# Autodesk Inventor assembly: Rail_AssemblyV2_0
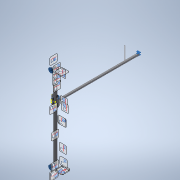
[picture p0: Inventor's stored thumbnail of the model, 180x180]
Saved by Autodesk Inventor 2021 (Build 250183000, 183)
## iProperties
Created: 2021-01-25
Part Number: Rail_AssemblyV2_0
Document SubType Name: Assembly
Designer: Jorian Brusind
Mass: 3786.54 g
Surface Area: 19508.5 cm^2
Volume: 2323.9 cm^3
Density: 1.62939 g/cm^3
Author: Jorian Brusind
## Documents named in this file (33)
- C:\Users\Jorian Brusind\Documents\GitHub\PersonalProjects\HyperRail\Inventor Files\Rail_AssemblyV2_0.iam
- C:\Users\Jorian Brusind\Documents\GitHub\PersonalProjects\Inventor Projects\Useful models\NEMA_Steppers\NEMA23\23HS8430B.ipt
- C:\Users\Jorian Brusind\Documents\GitHub\PersonalProjects\HyperRail\Inventor Files\NEMA23_StepperonlineMount.ipt
- C:\Users\Jorian Brusind\Documents\GitHub\PersonalProjects\Inventor Projects\Useful models\8020_Sets\IPT_20_Series\IPT_20_Series\20-2040_200mm.ipt
- C:\Users\Jorian Brusind\Documents\GitHub\PersonalProjects\HyperRail\Inventor Files\2804S_NEMA2115_1Gearbox.ipt
- C:\Users\Jorian Brusind\Documents\GitHub\PersonalProjects\HyperRail\PCB Files\Integrated Stepper Motor Driver\ExportSTEP\Main.iam
- C:\Users\Jorian Brusind\Documents\GitHub\PersonalProjects\HyperRail\Inventor Files\NEMA23_Shroud.ipt
- C:\Users\Jorian Brusind\Documents\GitHub\PersonalProjects\Inventor Projects\Useful models\8020_Sets\IPT_20_Series\IPT_20_Series\20-4040_2m.ipt
- C:\Users\Jorian Brusind\Documents\GitHub\PersonalProjects\HyperRail\Inventor Files\98952A059_ALUM MALE-FEM THRDED HEX STANDOFF.ipt
- C:\Users\Jorian Brusind\Documents\GitHub\PersonalProjects\HyperRail\Inventor Files\95783A039_NYLON 6-6 MALE-FEM THRDED HEX STANDOFF.ipt
- C:\Users\Jorian Brusind\Documents\GitHub\PersonalProjects\HyperRail\Inventor Files\Integrated_Stepper_NEMA23_Mount.ipt
- C:\Users\Jorian Brusind\Documents\GitHub\PersonalProjects\HyperRail\Inventor Files\Foot_Spacer.ipt
- C:\Users\Jorian Brusind\Documents\GitHub\PersonalProjects\Inventor Projects\Useful models\Metric bolt\Bolt M5 50mm.ipt
- C:\Users\Jorian Brusind\Documents\GitHub\PersonalProjects\Inventor Projects\Useful models\Metric nuts\Nut M5.ipt
- C:\Users\Jorian Brusind\Documents\GitHub\PersonalProjects\HyperRail\Inventor Files\Bottom_Foot.ipt
- C:\Users\Jorian Brusind\Documents\GitHub\PersonalProjects\HyperRail\Inventor Files\90deg_4040Bracket.ipt
- C:\Users\Jorian Brusind\Documents\GitHub\PersonalProjects\HyperRail\Inventor Files\X_Carriage_V2_0.iam
- C:\Users\Jorian Brusind\Documents\GitHub\PersonalProjects\Inventor Projects\Useful models\8020_Sets\IPT_40_Series\Extra_40_Series\HFS5-4060-4000\HFS5-4060-2125.ipt
- C:\Users\Jorian Brusind\Documents\GitHub\PersonalProjects\Inventor Projects\Useful models\8020_Sets\IPT_20_Series\IPT_20_Series\20-2040_150mm.ipt
- C:\Users\Jorian Brusind\Documents\GitHub\PersonalProjects\HyperRail\Inventor Files\RightAngle_Bracket_60mm.ipt
- C:\Users\Jorian Brusind\Documents\GitHub\PersonalProjects\Inventor Projects\Useful models\e2-micro-e-chains-small-and-lightweight-e-chains\03_07_012_0_160_5.iam
- C:\Users\Jorian Brusind\Documents\GitHub\PersonalProjects\HyperRail\Inventor Files\Cable_Guide_End.ipt
- C:\Users\Jorian Brusind\Documents\GitHub\PersonalProjects\Inventor Projects\Useful models\8020_Sets\AIS2018\20-2568_d.iam
- C:\Users\Jorian Brusind\Documents\GitHub\PersonalProjects\HyperRail\Inventor Files\5mm_bore_10mm_width_idlepulley.ipt
- C:\Users\Jorian Brusind\Documents\GitHub\PersonalProjects\HyperRail\Inventor Files\Idler_Spacer.ipt
- C:\Users\Jorian Brusind\Documents\GitHub\PersonalProjects\HyperRail\Inventor Files\Tape_Belt_Layer.ipt
- C:\Users\Jorian Brusind\Documents\GitHub\PersonalProjects\HyperRail\Inventor Files\SDP_sdpsi_a_6a55m028df0912\SDP_sdpsi_a_6a55m028df0912.ipt
- C:\Users\Jorian Brusind\Documents\GitHub\PersonalProjects\HyperRail\Inventor Files\X_CarriageR_V2_0.iam
- C:\Users\Jorian Brusind\Documents\GitHub\PersonalProjects\HyperRail\Inventor Files\X_CarriageL_V2_0_Short.iam
- C:\Users\Jorian Brusind\Documents\GitHub\PersonalProjects\HyperRail\Inventor Files\X_CarriageR_V2_0_Short.iam
- C:\Users\Jorian Brusind\Documents\GitHub\PersonalProjects\HyperRail\Inventor Files\SDP_sdpsi_a_6r25mc250\SDP_sdpsi_a_6r25mc1000.ipt
- C:\Users\Jorian Brusind\Documents\GitHub\PersonalProjects\Inventor Projects\Useful models\8020_Sets\IPT_20_Series\Extra_20_Series\8020_14056m\14056_m.ipt
- C:\Users\Jorian Brusind\Documents\GitHub\PersonalProjects\HyperRail\Inventor Files\Cable_Guide_Holder.ipt
## Components (51 placed, 32 different names)
1. 23HS8430B:1 — Mate:127, Angle:3, Mate:158, Mate:177, Mate:179, Mate:180, Mate:181, Mate:182, Mate:183, Mate:184, Mate:185, Mate:264, Mate:265, Mate:295
2. NEMA23_StepperonlineMount:1 — Angle:2, Mate:98, Mate:128, Mate:289, Flush:99, Mate:303, Mate:304, Flush:107, Flush:108
3. 20-2040_200mm:1 — Flush:88, Mate:284, Mate:301, Mate:302, Flush:111, Mate:334, Flush:125, Mate:335, Mate:337, Flush:127, Mate:338
4. 2804S_NEMA2115_1Gearbox:1 — Angle:2, Mate:98, Mate:127, Mate:128, Angle:3, Mate:158, Flush:86, Mate:336, Flush:126
5. Main:1 [sub-assembly] — Mate:291, Mate:292, Mate:293
6. 20-4040_2m:2 — Mate:232, Flush:73, Mate:233, Mate:234, Flush:74, Mate:288, Flush:98, Flush:123, Mate:322, Mate:323, Mate:326, Mate:327, Mate:330, Mate:331, Flush:124, Mate:345, Mate:346
7. NEMA23_Shroud:1 — Mate:264, Mate:265, Flush:86, Mate:294
8. 98952A059_ALUM MALE-FEM THRDED HEX STANDOFF:1 — Mate:180, Mate:181, Mate:186, Mate:191
9. 98952A059_ALUM MALE-FEM THRDED HEX STANDOFF:2 — Mate:184, Mate:185, Mate:189, Mate:192
10. 98952A059_ALUM MALE-FEM THRDED HEX STANDOFF:3 — Mate:177, Mate:179, Mate:187, Mate:190
11. 98952A059_ALUM MALE-FEM THRDED HEX STANDOFF:4 — Mate:182, Mate:183, Mate:188, Mate:193
12. 95783A039_NYLON 6-6 MALE-FEM THRDED HEX STANDOFF:1 — Mate:188, Mate:193
13. 95783A039_NYLON 6-6 MALE-FEM THRDED HEX STANDOFF:2 — Mate:186, Mate:191
14. 95783A039_NYLON 6-6 MALE-FEM THRDED HEX STANDOFF:3 — Mate:187, Mate:190
15. 95783A039_NYLON 6-6 MALE-FEM THRDED HEX STANDOFF:4 — Mate:189, Mate:192
16. Bolt M5 50mm:1 — Mate:224, Mate:245, Mate:246, Mate:247, Mate:269
17. Nut M5:1 — Mate:226, Mate:247
18. Nut M5:2 — Mate:244, Flush:78, Mate:246
19. Bottom_Foot:1 — Mate:224, Mate:226, Mate:245, Flush:81, Flush:93
20. 90deg_4040Bracket:1 — Mate:232, Flush:73, Mate:233, Flush:75
21. 90deg_4040Bracket:2 — Mate:234, Flush:74, Flush:75
22. Foot_Spacer:1 — Mate:244, Flush:78, Mate:269, Mate:283, Flush:94
23. Foot_Spacer:2 — Mate:250, Mate:281, Flush:91, Flush:92, Mate:282
24. Bottom_Foot:2 — Mate:249, Mate:251, Flush:81, Flush:93
25. Bolt M5 50mm:2 — Mate:249, Mate:250, Mate:251, Mate:282
26. 20-2040_200mm:2 — Flush:88, Mate:286, Flush:96, Flush:111, Flush:114, Flush:116, Mate:316, Flush:117, Flush:124, Mate:339, Flush:128, Mate:340, Mate:341, Flush:129, Mate:342
27. HFS5-4060-2125:1 — Mate:277, Mate:278, Mate:279, Mate:280, Mate:281, Flush:91, Flush:92, Mate:283, Flush:94, Mate:284, Flush:114, Mate:313, Flush:115, Mate:332, Mate:333, Mate:344, Flush:132, Flush:133, Mate:347, Mate:348, Mate:349, Flush:141, Flush:142
28. 20-2040_150mm:1 — Mate:286, Flush:96, Mate:288, Flush:98, Mate:289, Flush:99, Flush:138, Mate:352, Flush:139, Mate:353
29. Integrated_Stepper_NEMA23_Mount:1 — Mate:291, Mate:292, Mate:293, Mate:294, Mate:295
30. RightAngle_Bracket_60mm:1 — Mate:301, Mate:304, Flush:107
31. RightAngle_Bracket_60mm:2 — Mate:302, Mate:303, Flush:108
32. 03_07_012_0_160_5:1 [sub-assembly] — Mate:313, Flush:115, Mate:320
33. Cable_Guide_End:1 — Flush:116, Mate:316, Flush:117, Mate:320
34. 20-2568_d:1 [sub-assembly] — Flush:123, Mate:322, Mate:323
35. 5mm_bore_10mm_width_idlepulley:1 — Mate:324, Mate:325, Angle:4
36. Idler_Spacer:1 — Mate:324, Mate:325, Mate:326, Mate:327
37. 5mm_bore_10mm_width_idlepulley:2 — Mate:328, Mate:329, Angle:4
38. Idler_Spacer:2 — Mate:328, Mate:329, Mate:330, Mate:331
39. Tape_Belt_Layer:1 — Mate:332, Mate:333
40. X_Carriage_V2_0:1 [sub-assembly] — Mate:334, Flush:125, Mate:335
41. SDP_sdpsi_a_6a55m028df0912:1 — Mate:336, Flush:126
42. X_CarriageR_V2_0:1 [sub-assembly] — Mate:337, Flush:127, Mate:338
43. X_CarriageL_V2_0_Short:1 [sub-assembly] — Mate:341, Flush:129, Mate:342
44. X_CarriageR_V2_0_Short:1 [sub-assembly] — Mate:339, Flush:128, Mate:340
45. SDP_sdpsi_a_6r25mc1000:1 — Flush:130, Mate:343, Flush:131, Mate:344, Flush:132, Flush:133
46. SDP_sdpsi_a_6r25mc1000:2 — Flush:130, Mate:343, Flush:131
47. 14056_m:1 — Mate:346, Flush:138, Mate:352
48. 14056_m:3 — Mate:345, Flush:139, Mate:353
49. Cable_Guide_Holder:1 — Mate:348, Flush:136, Mate:350, Mate:351, Flush:140
50. Cable_Guide_Holder:2 — Mate:347, Mate:350, Flush:140, Flush:142
51. Cable_Guide_Holder:3 — Mate:349, Flush:136, Mate:351, Flush:141
## Relationships (131: Mate 90, Flush 38, Angle 3)
- Angle:2 (0 deg): NEMA23_StepperonlineMount:1 ↔ 2804S_NEMA2115_1Gearbox:1
- Mate:98: NEMA23_StepperonlineMount:1 ↔ 2804S_NEMA2115_1Gearbox:1
- Mate:127: 23HS8430B:1 ↔ 2804S_NEMA2115_1Gearbox:1
- Mate:128: NEMA23_StepperonlineMount:1 ↔ 2804S_NEMA2115_1Gearbox:1
- Angle:3 (0 deg): 23HS8430B:1 ↔ 2804S_NEMA2115_1Gearbox:1
- Mate:158: 23HS8430B:1 ↔ 2804S_NEMA2115_1Gearbox:1
- Mate:177: 23HS8430B:1 ↔ 98952A059_ALUM MALE-FEM THRDED HEX STANDOFF:3
- Mate:179: 23HS8430B:1 ↔ 98952A059_ALUM MALE-FEM THRDED HEX STANDOFF:3
- Mate:180: 23HS8430B:1 ↔ 98952A059_ALUM MALE-FEM THRDED HEX STANDOFF:1
- Mate:181: 23HS8430B:1 ↔ 98952A059_ALUM MALE-FEM THRDED HEX STANDOFF:1
- Mate:182: 23HS8430B:1 ↔ 98952A059_ALUM MALE-FEM THRDED HEX STANDOFF:4
- Mate:183: 23HS8430B:1 ↔ 98952A059_ALUM MALE-FEM THRDED HEX STANDOFF:4
- Mate:184: 23HS8430B:1 ↔ 98952A059_ALUM MALE-FEM THRDED HEX STANDOFF:2
- Mate:185: 23HS8430B:1 ↔ 98952A059_ALUM MALE-FEM THRDED HEX STANDOFF:2
- Mate:186: 98952A059_ALUM MALE-FEM THRDED HEX STANDOFF:1 ↔ 95783A039_NYLON 6-6 MALE-FEM THRDED HEX STANDOFF:2
- Mate:187: 98952A059_ALUM MALE-FEM THRDED HEX STANDOFF:3 ↔ 95783A039_NYLON 6-6 MALE-FEM THRDED HEX STANDOFF:3
- Mate:188: 98952A059_ALUM MALE-FEM THRDED HEX STANDOFF:4 ↔ 95783A039_NYLON 6-6 MALE-FEM THRDED HEX STANDOFF:1
- Mate:189: 98952A059_ALUM MALE-FEM THRDED HEX STANDOFF:2 ↔ 95783A039_NYLON 6-6 MALE-FEM THRDED HEX STANDOFF:4
- Mate:190: 98952A059_ALUM MALE-FEM THRDED HEX STANDOFF:3 ↔ 95783A039_NYLON 6-6 MALE-FEM THRDED HEX STANDOFF:3
- Mate:191: 98952A059_ALUM MALE-FEM THRDED HEX STANDOFF:1 ↔ 95783A039_NYLON 6-6 MALE-FEM THRDED HEX STANDOFF:2
- Mate:192: 98952A059_ALUM MALE-FEM THRDED HEX STANDOFF:2 ↔ 95783A039_NYLON 6-6 MALE-FEM THRDED HEX STANDOFF:4
- Mate:193: 98952A059_ALUM MALE-FEM THRDED HEX STANDOFF:4 ↔ 95783A039_NYLON 6-6 MALE-FEM THRDED HEX STANDOFF:1
- Mate:224: Bolt M5 50mm:1 ↔ Bottom_Foot:1
- Mate:226: Nut M5:1 ↔ Bottom_Foot:1
- Mate:232: 20-4040_2m:2 ↔ 90deg_4040Bracket:1
- Flush:73: 20-4040_2m:2 ↔ 90deg_4040Bracket:1
- Mate:233: 20-4040_2m:2 ↔ 90deg_4040Bracket:1
- Mate:234: 20-4040_2m:2 ↔ 90deg_4040Bracket:2
- Flush:74: 20-4040_2m:2 ↔ 90deg_4040Bracket:2
- Flush:75: 90deg_4040Bracket:1 ↔ 90deg_4040Bracket:2
- Mate:244: Nut M5:2 ↔ Foot_Spacer:1
- Flush:78: Nut M5:2 ↔ Foot_Spacer:1
- Mate:245: Bolt M5 50mm:1 ↔ Bottom_Foot:1
- Mate:246: Bolt M5 50mm:1 ↔ Nut M5:2
- Mate:247: Bolt M5 50mm:1 ↔ Nut M5:1
- Mate:249: Bottom_Foot:2 ↔ Bolt M5 50mm:2
- Mate:250: Foot_Spacer:2 ↔ Bolt M5 50mm:2
- Mate:251: Bottom_Foot:2 ↔ Bolt M5 50mm:2
- Flush:81: Bottom_Foot:1 ↔ Bottom_Foot:2
- Mate:264 (1 mm): 23HS8430B:1 ↔ NEMA23_Shroud:1
- Mate:265 (1 mm): 23HS8430B:1 ↔ NEMA23_Shroud:1
- Mate:269: Bolt M5 50mm:1 ↔ Foot_Spacer:1
- Flush:86: 2804S_NEMA2115_1Gearbox:1 ↔ NEMA23_Shroud:1
- Flush:88: 20-2040_200mm:1 ↔ 20-2040_200mm:2
- Mate:277: HFS5-4060-2125:1
- Mate:278: HFS5-4060-2125:1
- Mate:279: HFS5-4060-2125:1
- Mate:280: HFS5-4060-2125:1
- Mate:281: Foot_Spacer:2 ↔ HFS5-4060-2125:1
- Flush:91: Foot_Spacer:2 ↔ HFS5-4060-2125:1
- Flush:92 (20 mm): Foot_Spacer:2 ↔ HFS5-4060-2125:1
- Mate:282: Foot_Spacer:2 ↔ Bolt M5 50mm:2
- Flush:93: Bottom_Foot:1 ↔ Bottom_Foot:2
- Mate:283 (-40 mm): Foot_Spacer:1 ↔ HFS5-4060-2125:1
- Flush:94: Foot_Spacer:1 ↔ HFS5-4060-2125:1
- Mate:284 (24 mm): 20-2040_200mm:1 ↔ HFS5-4060-2125:1
- Mate:286: 20-2040_200mm:2 ↔ 20-2040_150mm:1
- Flush:96 (-5 mm): 20-2040_200mm:2 ↔ 20-2040_150mm:1
- Mate:288: 20-4040_2m:2 ↔ 20-2040_150mm:1
- Flush:98: 20-4040_2m:2 ↔ 20-2040_150mm:1
- Mate:289 (10 mm): NEMA23_StepperonlineMount:1 ↔ 20-2040_150mm:1
- Flush:99 (-12.5 mm): NEMA23_StepperonlineMount:1 ↔ 20-2040_150mm:1
- Mate:291: Main:1 ↔ Integrated_Stepper_NEMA23_Mount:1
- Mate:292: Main:1 ↔ Integrated_Stepper_NEMA23_Mount:1
- Mate:293: Main:1 ↔ Integrated_Stepper_NEMA23_Mount:1
- Mate:294: NEMA23_Shroud:1 ↔ Integrated_Stepper_NEMA23_Mount:1
- Mate:295: 23HS8430B:1 ↔ Integrated_Stepper_NEMA23_Mount:1
- Mate:301: 20-2040_200mm:1 ↔ RightAngle_Bracket_60mm:1
- Mate:302: 20-2040_200mm:1 ↔ RightAngle_Bracket_60mm:2
- Mate:303: NEMA23_StepperonlineMount:1 ↔ RightAngle_Bracket_60mm:2
- Mate:304: NEMA23_StepperonlineMount:1 ↔ RightAngle_Bracket_60mm:1
- Flush:107: NEMA23_StepperonlineMount:1 ↔ RightAngle_Bracket_60mm:1
- Flush:108: NEMA23_StepperonlineMount:1 ↔ RightAngle_Bracket_60mm:2
- Flush:111: 20-2040_200mm:1 ↔ 20-2040_200mm:2
- Flush:114: 20-2040_200mm:2 ↔ HFS5-4060-2125:1
- Mate:313 (2 mm): HFS5-4060-2125:1 ↔ 03_07_012_0_160_5:1
- Flush:115: HFS5-4060-2125:1 ↔ 03_07_012_0_160_5:1
- Flush:116: 20-2040_200mm:2 ↔ Cable_Guide_End:1
- Mate:316: 20-2040_200mm:2 ↔ Cable_Guide_End:1
- Flush:117: 20-2040_200mm:2 ↔ Cable_Guide_End:1
- Mate:320: 03_07_012_0_160_5:1 ↔ Cable_Guide_End:1
- Flush:123: 20-4040_2m:2 ↔ 20-2568_d:1
- Mate:322 (-2 mm): 20-4040_2m:2 ↔ 20-2568_d:1
- Mate:323: 20-4040_2m:2 ↔ 20-2568_d:1
- Mate:324: 5mm_bore_10mm_width_idlepulley:1 ↔ Idler_Spacer:1
- Mate:325: 5mm_bore_10mm_width_idlepulley:1 ↔ Idler_Spacer:1
- Mate:326: 20-4040_2m:2 ↔ Idler_Spacer:1
- Mate:327 (2.5 mm): 20-4040_2m:2 ↔ Idler_Spacer:1
- Mate:328: 5mm_bore_10mm_width_idlepulley:2 ↔ Idler_Spacer:2
- Mate:329: 5mm_bore_10mm_width_idlepulley:2 ↔ Idler_Spacer:2
- Mate:330: 20-4040_2m:2 ↔ Idler_Spacer:2
- Mate:331 (2.5 mm): 20-4040_2m:2 ↔ Idler_Spacer:2
- Angle:4 (0 deg): 5mm_bore_10mm_width_idlepulley:1 ↔ 5mm_bore_10mm_width_idlepulley:2
- Flush:124 (32 mm): 20-4040_2m:2 ↔ 20-2040_200mm:2
- Mate:332: HFS5-4060-2125:1 ↔ Tape_Belt_Layer:1
- Mate:333 (1 mm): HFS5-4060-2125:1 ↔ Tape_Belt_Layer:1
- Mate:334: 20-2040_200mm:1 ↔ X_Carriage_V2_0:1
- Flush:125: 20-2040_200mm:1 ↔ X_Carriage_V2_0:1
- Mate:335 (5 mm): 20-2040_200mm:1 ↔ X_Carriage_V2_0:1
- Mate:336: 2804S_NEMA2115_1Gearbox:1 ↔ SDP_sdpsi_a_6a55m028df0912:1
- Flush:126: 2804S_NEMA2115_1Gearbox:1 ↔ SDP_sdpsi_a_6a55m028df0912:1
- Mate:337: 20-2040_200mm:1 ↔ X_CarriageR_V2_0:1
- Flush:127: 20-2040_200mm:1 ↔ X_CarriageR_V2_0:1
- Mate:338 (5 mm): 20-2040_200mm:1 ↔ X_CarriageR_V2_0:1
- Mate:339: 20-2040_200mm:2 ↔ X_CarriageR_V2_0_Short:1
- Flush:128: 20-2040_200mm:2 ↔ X_CarriageR_V2_0_Short:1
- Mate:340 (7 mm): 20-2040_200mm:2 ↔ X_CarriageR_V2_0_Short:1
- Mate:341: 20-2040_200mm:2 ↔ X_CarriageL_V2_0_Short:1
- Flush:129: 20-2040_200mm:2 ↔ X_CarriageL_V2_0_Short:1
- Mate:342 (7 mm): 20-2040_200mm:2 ↔ X_CarriageL_V2_0_Short:1
- Flush:130: SDP_sdpsi_a_6r25mc1000:1 ↔ SDP_sdpsi_a_6r25mc1000:2
- Mate:343: SDP_sdpsi_a_6r25mc1000:1 ↔ SDP_sdpsi_a_6r25mc1000:2
- Flush:131: SDP_sdpsi_a_6r25mc1000:1 ↔ SDP_sdpsi_a_6r25mc1000:2
- Mate:344 (1 mm): HFS5-4060-2125:1 ↔ SDP_sdpsi_a_6r25mc1000:1
- Flush:132: HFS5-4060-2125:1 ↔ SDP_sdpsi_a_6r25mc1000:1
- Flush:133: HFS5-4060-2125:1 ↔ SDP_sdpsi_a_6r25mc1000:1
- Mate:345: 20-4040_2m:2 ↔ 14056_m:3
- Mate:346: 20-4040_2m:2 ↔ 14056_m:1
- Mate:347: HFS5-4060-2125:1 ↔ Cable_Guide_Holder:2
- Mate:348: HFS5-4060-2125:1 ↔ Cable_Guide_Holder:1
- Mate:349: HFS5-4060-2125:1 ↔ Cable_Guide_Holder:3
- Flush:136: Cable_Guide_Holder:1 ↔ Cable_Guide_Holder:3
- Mate:350 (100 mm): Cable_Guide_Holder:1 ↔ Cable_Guide_Holder:2
- Mate:351 (100 mm): Cable_Guide_Holder:1 ↔ Cable_Guide_Holder:3
- Flush:138: 20-2040_150mm:1 ↔ 14056_m:1
- Mate:352: 20-2040_150mm:1 ↔ 14056_m:1
- Flush:139: 20-2040_150mm:1 ↔ 14056_m:3
- Mate:353: 20-2040_150mm:1 ↔ 14056_m:3
- Flush:140: Cable_Guide_Holder:1 ↔ Cable_Guide_Holder:2
- Flush:141: HFS5-4060-2125:1 ↔ Cable_Guide_Holder:3
- Flush:142 (200 mm): HFS5-4060-2125:1 ↔ Cable_Guide_Holder:2
